# Autodesk Inventor assembly: Assembly1
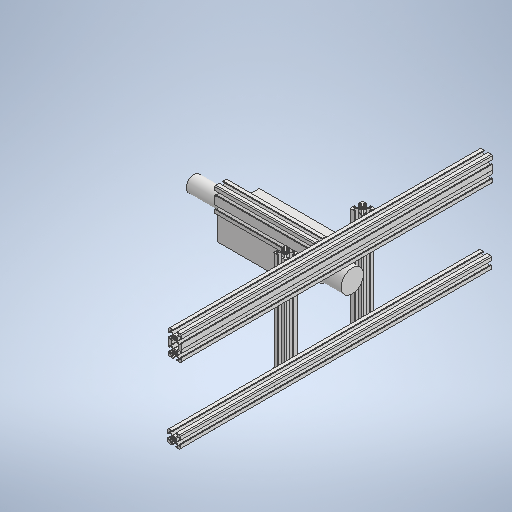
[picture p0: Inventor's stored thumbnail of the model, 512x512]
Saved by Autodesk Inventor 2026.2 (Build 302298000, 298)
## iProperties
Created: 2026-04-09
Part Number: Assembly1
Document SubType Name: Assembly
Designer: mumin
Author: mumin
## Documents named in this file (7)
- C:\GitHub\In-situ-monitoring-of-powder-bed-fusion-additive-manufacturing\accessories\Vibrometer Test Rig\Assembly1.iam
- C:\GitHub\In-situ-monitoring-of-powder-bed-fusion-additive-manufacturing\accessories\Vibrometer Test Rig\2040 Legs (500mm).ipt
- C:\GitHub\In-situ-monitoring-of-powder-bed-fusion-additive-manufacturing\accessories\Vibrometer Test Rig\2020 Legs (160mm).ipt
- C:\GitHub\In-situ-monitoring-of-powder-bed-fusion-additive-manufacturing\accessories\Vibrometer Test Rig\2020 Legs (500mm).ipt
- C:\GitHub\In-situ-monitoring-of-powder-bed-fusion-additive-manufacturing\accessories\Vibrometer Test Rig\2040 Legs (160mm).ipt
- C:\GitHub\In-situ-monitoring-of-powder-bed-fusion-additive-manufacturing\accessories\Vibrometer Test Rig\LV_Bracket_2.ipt
- C:\GitHub\In-situ-monitoring-of-powder-bed-fusion-additive-manufacturing\accessories\Vibrometer Test Rig\Updated Laser Scanner.ipt
## Components (7 placed, 6 different names)
1. 2040 Legs (500mm):1 — Flush:1, Mate:1, Flush:2, Mate:2, Mate:4, Flush:4
2. 2020 Legs (160mm):1 — Flush:1, Mate:1
3. 2020 Legs (160mm):2 — Flush:2, Mate:2, Flush:3, Mate:3
4. 2020 Legs (500mm):1 — Flush:3, Mate:3
5. 2040 Legs (160mm):1 — Mate:4, Flush:4, Flush:5, Mate:5
6. LV_Bracket_2:1 — Flush:5, Mate:5, Insert:1, Insert:2
7. Updated Laser Scanner:1 — Insert:1, Insert:2
## Relationships (12: Flush 5, Mate 5, Insert 2)
- Flush:1: 2040 Legs (500mm):1 ↔ 2020 Legs (160mm):1
- Mate:1: 2040 Legs (500mm):1 ↔ 2020 Legs (160mm):1
- Flush:2: 2040 Legs (500mm):1 ↔ 2020 Legs (160mm):2
- Mate:2: 2040 Legs (500mm):1 ↔ 2020 Legs (160mm):2
- Flush:3: 2020 Legs (160mm):2 ↔ 2020 Legs (500mm):1
- Mate:3: 2020 Legs (160mm):2 ↔ 2020 Legs (500mm):1
- Mate:4: 2040 Legs (500mm):1 ↔ 2040 Legs (160mm):1
- Flush:4: 2040 Legs (500mm):1 ↔ 2040 Legs (160mm):1
- Flush:5: 2040 Legs (160mm):1 ↔ LV_Bracket_2:1
- Mate:5: 2040 Legs (160mm):1 ↔ LV_Bracket_2:1
- Insert:1: LV_Bracket_2:1 ↔ Updated Laser Scanner:1
- Insert:2: LV_Bracket_2:1 ↔ Updated Laser Scanner:1
